# Autodesk Inventor assembly: 1-Post Hex Nut Retainer With Nylon Hardware
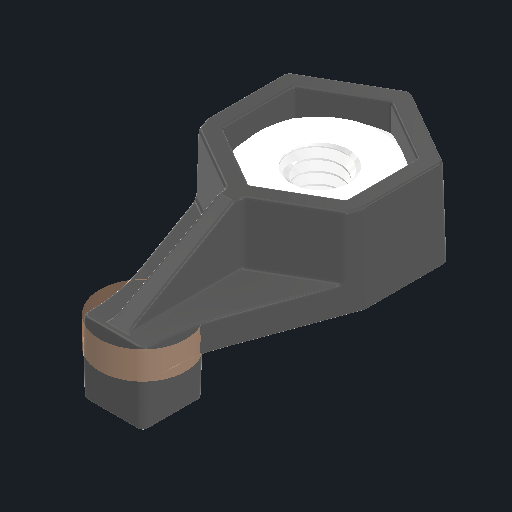
[picture p0: Inventor's stored thumbnail of the model, 512x512]
Saved by Autodesk Inventor 2025 (Build 290162000, 162)
## iProperties
Created: 2024-11-07
Part Number: 1-Post Hex Nut Retainer With Nylon Hardware
Document SubType Name: Assembly
Designer: avere
Author: avere
## Documents named in this file (4)
- D:\VEX\High Stakes\CAD\ROBOPROS-CAD-Inventor\Structure\1-Post Hex Nut Retainer With Nylon Hardware.iam
- D:\VEX\High Stakes\CAD\ROBOPROS-CAD-Inventor\Structure\1-Post Hex Nut Retainer.ipt
- D:\VEX\High Stakes\CAD\ROBOPROS-CAD-Inventor\Structure\Hardware\Nut Nylon\Nut Nylon - White.ipt
- C:\Users\avere\VEX\High Stakes\CAD\ROBOPROS-CAD-Inventor\Structure\Hardware\Nut Nylon.ipt
## Components (2 placed, 2 different names)
1. 1-Post Hex Nut Retainer:1 — Insert:1
2. Nut Nylon - White:1 — Insert:1
## Relationships (1: Insert 1)
- Insert:1: 1-Post Hex Nut Retainer:1 ↔ Nut Nylon - White:1
